# Autodesk Inventor assembly: Отсек электроники
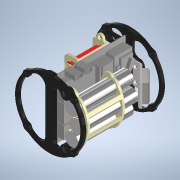
[picture p0: Inventor's stored thumbnail of the model, 180x180]
Saved by Autodesk Inventor 2022 (Build 260153000, 153)
## iProperties
Created: 2022-05-03
Part Number: Отсек электроники
Document SubType Name: Assembly
Designer: Кочетов.А.И.
Author: Кочетов.А.И.
## Documents named in this file (8)
- C:\Users\BornO\Desktop\Отсек электроники v0.1 ТТ-1\Отсек электроники.iam
- C:\Users\BornO\Desktop\Отсек электроники v0.1 ТТ-1\БАСУ\Нижнее крепление.ipt
- C:\Users\BornO\Desktop\Отсек электроники v0.1 ТТ-1\БАСУ\БАСУ.ipt
- C:\Users\BornO\Desktop\Отсек электроники v0.1 ТТ-1\БАСУ\Верхнее крепление.ipt
- C:\Users\BornO\Desktop\Отсек электроники v0.1 ТТ-1\РБАСУ\Сборка РБАСУ.iam
- C:\Users\BornO\Desktop\Отсек электроники v0.1 ТТ-1\АКБ\АКБ Сборка.iam
- C:\Users\BornO\Desktop\Отсек электроники v0.1 ТТ-1\GPS\GPS.ipt.iam
- GPS.ipt
## Components (6 placed, 6 different names)
1. Нижнее крепление:1 — Совмещение:1, Совмещение:2, Заподлицо:1, Совмещение:3, Совмещение:4, Совмещение:5, Совмещение:12, Совмещение:13, Совмещение:14
2. БАСУ:1 — Совмещение:3, Совмещение:4, Совмещение:5, Совмещение:6, Совмещение:7, Совмещение:8
3. Верхнее крепление:1 — Совмещение:6, Совмещение:7, Совмещение:8, Совмещение:9, Совмещение:10, Совмещение:11, Совмещение:15, Совмещение:16, Совмещение:17
4. Сборка РБАСУ:1 [sub-assembly] — Совмещение:9, Совмещение:10, Совмещение:11
5. АКБ Сборка:1 [sub-assembly] — Совмещение:12, Совмещение:13, Совмещение:14
6. GPS.ipt:1 [sub-assembly] — Совмещение:15, Совмещение:16, Совмещение:17
## Relationships (18: Mate 17, Flush 1)
- Совмещение:1 [Mate]: Нижнее крепление:1
- Совмещение:2 [Mate]: Нижнее крепление:1
- Заподлицо:1 [Flush]: Нижнее крепление:1
- Совмещение:3 [Mate]: Нижнее крепление:1 ↔ БАСУ:1
- Совмещение:4 [Mate]: Нижнее крепление:1 ↔ БАСУ:1
- Совмещение:5 [Mate]: Нижнее крепление:1 ↔ БАСУ:1
- Совмещение:6 [Mate]: БАСУ:1 ↔ Верхнее крепление:1
- Совмещение:7 [Mate]: БАСУ:1 ↔ Верхнее крепление:1
- Совмещение:8 [Mate]: БАСУ:1 ↔ Верхнее крепление:1
- Совмещение:9 [Mate]: Верхнее крепление:1 ↔ Сборка РБАСУ:1
- Совмещение:10 [Mate]: Верхнее крепление:1 ↔ Сборка РБАСУ:1
- Совмещение:11 [Mate]: Верхнее крепление:1 ↔ Сборка РБАСУ:1
- Совмещение:12 [Mate]: Нижнее крепление:1 ↔ АКБ Сборка:1
- Совмещение:13 [Mate]: Нижнее крепление:1 ↔ АКБ Сборка:1
- Совмещение:14 [Mate]: Нижнее крепление:1 ↔ АКБ Сборка:1
- Совмещение:15 [Mate]: Верхнее крепление:1 ↔ GPS.ipt:1
- Совмещение:16 [Mate]: Верхнее крепление:1 ↔ GPS.ipt:1
- Совмещение:17 [Mate]: Верхнее крепление:1 ↔ GPS.ipt:1
